# Autodesk Inventor assembly: Convery Digital Prototype
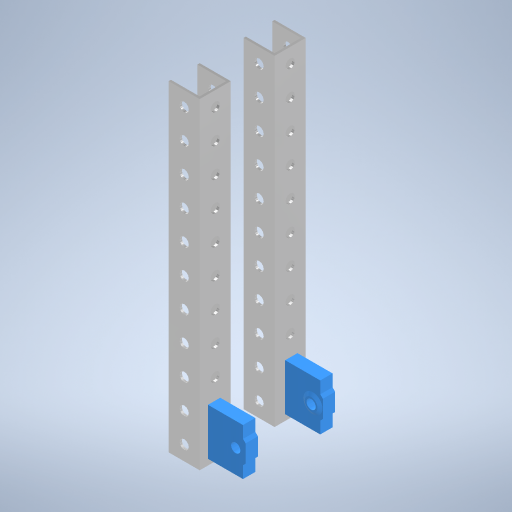
[picture p0: Inventor's stored thumbnail of the model, 512x512]
Saved by Autodesk Inventor 2024 (Build 280153020, 153B)
## iProperties
Created: 2024-02-06
Part Number: Convery Digital Prototype
Document SubType Name: Assembly
Designer: scottst
Author: scottst
## Documents named in this file (3)
- H:\Robotics Club\3D Models\Mr Scott\Convery Digital Prototype.iam
- H:\Robotics Club\3D Models\Mr Scott\C-Channel 11in.ipt
- H:\Robotics Club\3D Models\Mr Scott\Roller Bracket.ipt
## Components (4 placed, 2 different names)
1. C-Channel 11in:1 — Flush:1, Flush:2, Mate:2, Mate:3, Mate:4
2. C-Channel 11in:2 — Flush:1, Flush:2, Mate:1, Mate:5, Mate:6
3. Roller Bracket:1 — Mate:1, Mate:5, Mate:6
4. Roller Bracket:2 — Mate:2, Mate:3, Mate:4
## Relationships (8: Mate 6, Flush 2)
- Flush:1: C-Channel 11in:1 ↔ C-Channel 11in:2
- Flush:2: C-Channel 11in:1 ↔ C-Channel 11in:2
- Mate:1: C-Channel 11in:2 ↔ Roller Bracket:1
- Mate:2: C-Channel 11in:1 ↔ Roller Bracket:2
- Mate:3: C-Channel 11in:1 ↔ Roller Bracket:2
- Mate:4: C-Channel 11in:1 ↔ Roller Bracket:2
- Mate:5: C-Channel 11in:2 ↔ Roller Bracket:1
- Mate:6: C-Channel 11in:2 ↔ Roller Bracket:1
